# Autodesk Inventor assembly: TW1
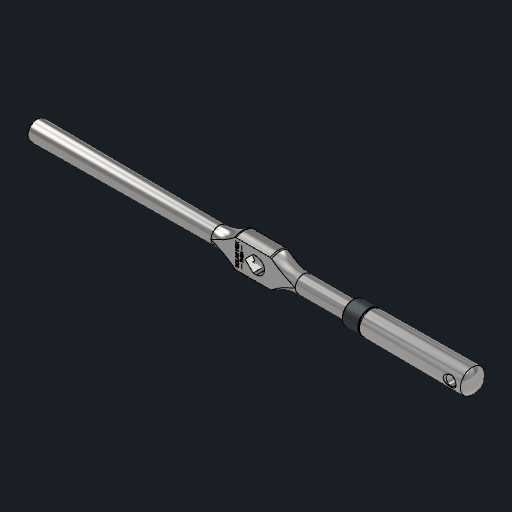
[picture p0: Inventor's stored thumbnail of the model, 512x512]
Saved by Autodesk Inventor 2025.3 (Build 293356000, 356)
## iProperties
Created: 2025-05-04
Part Number: TW1
Document SubType Name: Assembly
Designer: fablabadmin
Description: Tap wrench
Stock Number: -
Author: Benjamin Solar
Title: WEDU
Revision Number: 1
## Documents named in this file (7)
- C:\Users\fablabadmin\Documents\_Benjamin_S\_3dCAD\HHVerkstad\TapWrench2A\TW2A.iam
- C:\Users\fablabadmin\Documents\_Benjamin_S\_3dCAD\HHVerkstad\TapWrench2A\TW2A-001.ipt
- C:\Users\fablabadmin\Documents\_Benjamin_S\_3dCAD\HHVerkstad\TapWrench2A\TW2A-002.ipt
- C:\Users\fablabadmin\Documents\_Benjamin_S\_3dCAD\HHVerkstad\TapWrench2A\TW2A-003.ipt
- C:\Users\fablabadmin\Documents\_Benjamin_S\_3dCAD\HHVerkstad\TapWrench2A\TW2A-004A.ipt
- C:\Users\fablabadmin\Documents\_Benjamin_S\_3dCAD\HHVerkstad\TapWrench2A\E002M12.ipt
- C:\Users\fablabadmin\Documents\_Benjamin_S\_3dCAD\HHVerkstad\TapWrench2A\TW2A-004B.ipt
## Components (6 placed, 6 different names)
1. TW2A-001:1 — Mate:1, Angle:1, Mate:3, Mate:4, Mate:5, Mate:6, Mate:7, Mate:10, Mate:11
2. TW2A-002:1 — Mate:1, Angle:1, Mate:2, Tangent:1, Mate:8, Mate:10, Tangent:2
3. TW2A-003:1 — Mate:2, Mate:3
4. TW2A-004A:1 — Mate:4, Angle:2, Tangent:1
5. E002M12:1 — Mate:5, Mate:6, Mate:7, Mate:8
6. TW2A-004B:1 — Flush:1, Mate:11, Tangent:2
## Relationships (15: Mate 10, Angle 2, Tangent 2, Flush 1)
- Mate:1: TW2A-001:1 ↔ TW2A-002:1
- Angle:1 (0 deg): TW2A-001:1 ↔ TW2A-002:1
- Mate:2: TW2A-002:1 ↔ TW2A-003:1
- Mate:3: TW2A-001:1 ↔ TW2A-003:1
- Mate:4: TW2A-001:1 ↔ TW2A-004A:1
- Angle:2 (0 deg): TW2A-004A:1
- Tangent:1: TW2A-002:1 ↔ TW2A-004A:1
- Mate:5: TW2A-001:1 ↔ E002M12:1
- Mate:6: TW2A-001:1 ↔ E002M12:1
- Mate:7: TW2A-001:1 ↔ E002M12:1
- Mate:8: TW2A-002:1 ↔ E002M12:1
- Flush:1: TW2A-004B:1
- Mate:10: TW2A-001:1 ↔ TW2A-002:1
- Mate:11: TW2A-001:1 ↔ TW2A-004B:1
- Tangent:2: TW2A-002:1 ↔ TW2A-004B:1
